# Autodesk Inventor assembly: Сборка1
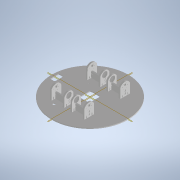
[picture p0: Inventor's stored thumbnail of the model, 180x180]
Saved by Autodesk Inventor 2020 (Build 240168000, 168)
## iProperties
Created: 2022-02-23
Part Number: Сборка1
Document SubType Name: Assembly
Designer: Dell
Author: Dell
## Documents named in this file (5)
- C:\Users\Dell\Desktop\OnStage\3D\Нижняя_платформа\Сборка1.iam
- C:\Users\Dell\Desktop\OnStage\3D\Нижняя_платформа\Нижний_круг_платформа.ipt
- C:\Users\Dell\Desktop\OnStage\3D\Нижняя_платформа\Крепление_мотора1_платформа.ipt
- C:\Users\Dell\Desktop\OnStage\3D\Нижняя_платформа\Крепление_мотора2_платформа.ipt
- C:\Users\Dell\Desktop\OnStage\3D\Нижняя_платформа\Крепление_мотора3_платформа.ipt
## Components (13 placed, 4 different names)
1. Нижний_круг_платформа:1
2. Крепление_мотора1_платформа:1
3. Крепление_мотора1_платформа:2
4. Крепление_мотора1_платформа:3
5. Крепление_мотора1_платформа:4
6. Крепление_мотора2_платформа:1
7. Крепление_мотора2_платформа:2
8. Крепление_мотора2_платформа:3
9. Крепление_мотора2_платформа:4
10. Крепление_мотора3_платформа:1
11. Крепление_мотора3_платформа:2
12. Крепление_мотора3_платформа:3
13. Крепление_мотора3_платформа:4
## Component patterns: (4 elements, first: Крепление_мотора1_платформа:1), (4 elements, first: Крепление_мотора2_платформа:1), (4 elements, first: Крепление_мотора3_платформа:1)
